# Autodesk Inventor assembly: Y-Shafts-Holder
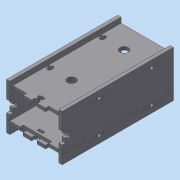
[picture p0: Inventor's stored thumbnail of the model, 180x180]
Saved by Autodesk Inventor 2016 SP1 (Build 200210100, 210)
## iProperties
Created: 2016-01-21
Part Number: Y-Shafts-Holder
Document SubType Name: Assembly
Designer: Mohamed A.
Author: Mohamed A.
## Documents named in this file (4)
- C:\Users\Mohamed\Documents\inventor\StemCellsPlatform\Laser Cut\Y-Shafts-Holder\Y-Shafts-Holder.iam
- C:\Users\Mohamed\Documents\inventor\StemCellsPlatform\Laser Cut\Y-Shafts-Holder\Y-Shafts-Holder_Front-Outer.ipt
- C:\Users\Mohamed\Documents\inventor\StemCellsPlatform\Laser Cut\Y-Shafts-Holder\Y-Shafts-Holder_Front-Inner.ipt
- C:\Users\Mohamed\Documents\inventor\StemCellsPlatform\Laser Cut\Y-Shafts-Holder\Y-Shafts-Holder_Side.ipt
## Components (5 placed, 3 different names)
1. Y-Shafts-Holder_Front-Outer:1 — Mate:1, Flush:1, Flush:2, Flush:3, Flush:4, Mate:2, Flush:8, Flush:9, Flush:10, Flush:11, Flush:12
2. Y-Shafts-Holder_Front-Inner:1 — Mate:1, Flush:1, Flush:2
3. Y-Shafts-Holder_Front-Outer:2 — Flush:3, Flush:4, Mate:2, Flush:15
4. Y-Shafts-Holder_Side:1 — Flush:9, Flush:11, Flush:12, Flush:13, Flush:14
5. Y-Shafts-Holder_Side:2 — Flush:8, Flush:10, Flush:13, Flush:14, Flush:15
## Relationships (14: Flush 12, Mate 2)
- Mate:1: Y-Shafts-Holder_Front-Outer:1 ↔ Y-Shafts-Holder_Front-Inner:1
- Flush:1: Y-Shafts-Holder_Front-Outer:1 ↔ Y-Shafts-Holder_Front-Inner:1
- Flush:2: Y-Shafts-Holder_Front-Outer:1 ↔ Y-Shafts-Holder_Front-Inner:1
- Flush:3: Y-Shafts-Holder_Front-Outer:1 ↔ Y-Shafts-Holder_Front-Outer:2
- Flush:4: Y-Shafts-Holder_Front-Outer:1 ↔ Y-Shafts-Holder_Front-Outer:2
- Mate:2 (-33 mm): Y-Shafts-Holder_Front-Outer:1 ↔ Y-Shafts-Holder_Front-Outer:2
- Flush:8: Y-Shafts-Holder_Front-Outer:1 ↔ Y-Shafts-Holder_Side:2
- Flush:9: Y-Shafts-Holder_Front-Outer:1 ↔ Y-Shafts-Holder_Side:1
- Flush:10: Y-Shafts-Holder_Front-Outer:1 ↔ Y-Shafts-Holder_Side:2
- Flush:11: Y-Shafts-Holder_Front-Outer:1 ↔ Y-Shafts-Holder_Side:1
- Flush:12 (-5 mm): Y-Shafts-Holder_Front-Outer:1 ↔ Y-Shafts-Holder_Side:1
- Flush:13: Y-Shafts-Holder_Side:1 ↔ Y-Shafts-Holder_Side:2
- Flush:14: Y-Shafts-Holder_Side:1 ↔ Y-Shafts-Holder_Side:2
- Flush:15: Y-Shafts-Holder_Front-Outer:2 ↔ Y-Shafts-Holder_Side:2
